# Autodesk Inventor assembly: a1614chal
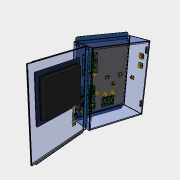
[picture p0: Inventor's stored thumbnail of the model, 180x180]
Saved by Autodesk Inventor 2020.1 (Build 241239000, 239)
## iProperties
Created: 2009-10-15
Part Number: a1614chal
Document SubType Name: Assembly
Designer: Thom Tremblay
Translation Standard: STEP AP214IS
FileName: a1614chal.STEP
PreProcessor: SolidWorks 2007
PostProcessor: Build: 253, Release: 2010 SP1 - Date: Wed 07/29/2009
Sent Units: inch
Uncertainty: 1e-05
Author: Thom Tremblay
## Documents named in this file (20)
- C:\Users\thom_tremblay\Desktop\Inventor ACP prep data\Week 1\Electrical Enclosure.iam
- C:\Users\thom_tremblay\Desktop\Inventor ACP prep data\Week 1\Electrical Enclosure\Clamp.ipt
- C:\Users\thom_tremblay\Desktop\Inventor ACP prep data\Week 1\Electrical Enclosure\Housing.iam
- C:\Users\thom_tremblay\Desktop\Inventor ACP prep data\Week 1\Electrical Enclosure\Panel_CHJunction_16x14.ipt
- C:\Users\thom_tremblay\Desktop\Inventor ACP prep data\Week 1\Electrical Enclosure\Cover.iam
- C:\Users\thom_tremblay\Desktop\Inventor ACP prep data\Week 1\Electrical Enclosure\Control Panel.ipt
- C:\Users\thom_tremblay\Desktop\Inventor ACP prep data\Week 1\Electrical Enclosure\Ribbon Tape.ipt
- C:\Users\thom_tremblay\Desktop\Inventor ACP prep data\Week 1\Electrical Enclosure\ribbon cable connector.ipt
- C:\Users\thom_tremblay\Desktop\Inventor ACP prep data\Week 1\Electrical Enclosure\Hinge.iam
- C:\Users\thom_tremblay\Desktop\Inventor ACP prep data\Week 1\Electrical Enclosure\Cable Mount.iam
- C:\Users\thom_tremblay\Desktop\Inventor ACP prep data\Week 1\Electrical Enclosure\Communication PCB.ipt
- C:\Users\thom_tremblay\Desktop\Inventor ACP prep data\Week 1\Electrical Enclosure\Graphics.iam
- C:\Users\thom_tremblay\Desktop\Inventor ACP prep data\Week 1\Electrical Enclosure\CPU_PCB.ipt
- C:\Users\thom_tremblay\Desktop\Inventor ACP prep data\Week 1\Electrical Enclosure\8 Pin Header.ipt
- C:\Users\thom_tremblay\Desktop\Inventor ACP prep data\Week 1\Electrical Enclosure\Connector, IDC, 8 Pin, SR.ipt
- C:\Users\thom_tremblay\Desktop\Inventor ACP prep data\Week 1\Electrical Enclosure\360124.ipt
- C:\Users\thom_tremblay\Desktop\Inventor ACP prep data\Week 1\Electrical Enclosure\12 Pin DR.ipt
- C:\Users\thom_tremblay\Desktop\Inventor ACP prep data\Week 1\Electrical Enclosure\RC Male Connector.ipt
- C:\Users\thom_tremblay\Desktop\Inventor ACP prep data\Week 1\Electrical Enclosure\DB9 Female.ipt
- C:\Users\thom_tremblay\Desktop\Inventor ACP prep data\Week 1\Electrical Enclosure\10 Pin DR.ipt
## Components (29 placed, 19 different names)
1. Clamp:1
2. Housing:1 [sub-assembly] — Insert:1, Angle:1, Mate:5, Mate:6, Mate:7, Flush:7, Mate:13, Mate:22, Flush:17, Flush:20, Insert:3, Angle:6, Mate:29, Flush:32
3. Panel_CHJunction_16x14:1 — Insert:1, Angle:1, Angle:2, Mate:15, Angle:4, Mate:17, Flush:8, Flush:9, Flush:10, Flush:11, Mate:18, Flush:12, Flush:13, Mate:30, Flush:33, Mate:32, Mate:34
4. Clamp:2
5. Hinge:1 [sub-assembly] — Mate:16
6. Cover:1 [sub-assembly] — Flush:3, Mate:2, Mate:3, Mate:4, Mate:14, Angle:3
7. Control Panel:1 — Flush:3, Mate:2, Mate:3, Mate:9, Mate:10, Mate:11, Mate:28, Flush:30, Flush:31
8. Ribbon Tape:1 — Mate:5, Mate:6, Flush:4, Mate:7
9. Ribbon Tape:2 — Mate:4, Flush:4, Flush:7
10. ribbon cable connector:1 — Mate:9, Mate:10, Mate:11
11. Communication PCB:1 — Mate:15, Angle:4, Flush:10, Flush:11, Flush:21, Flush:22, Mate:25, Flush:25, Flush:26
12. DB9 Female:1
13. RC Male Connector:1
14. Graphics:1 [sub-assembly] — Mate:17, Flush:8, Flush:9, Mate:31, Flush:34, Flush:35
15. CPU_PCB:1 — Mate:18, Flush:12, Flush:13, Mate:19, Flush:14, Flush:15, Mate:33
16. 8 Pin Header:1 — Mate:19, Flush:14, Flush:15, Flush:16, Mate:21
17. Connector, IDC, 8 Pin, SR:1 — Flush:16, Mate:21
18. 360124:1 — Mate:22, Flush:17, Flush:20
19. 360124:2 — Insert:3, Angle:6
20. 12 Pin DR:2 — Mate:25, Flush:25, Flush:26
21. 10 Pin DR:2 — Flush:21, Flush:22
22. 10 Pin DR:1 — Mate:31, Flush:34, Flush:35
23. DB9 Female:2 — Mate:28, Flush:30, Flush:31
24. Cable Mount:1 [sub-assembly] — Mate:13, Angle:2
25. Cable Mount:2 [sub-assembly] — Mate:14, Angle:3, Mate:16
26. Cable Mount:3 [sub-assembly] — Mate:29, Flush:32
27. Cable Mount:4 [sub-assembly] — Mate:30, Flush:33
28. Cable Mount:5 [sub-assembly] — Mate:32, Mate:33, Flush:36
29. Cable Mount:6 [sub-assembly] — Mate:34, Flush:36
## Relationships (73: Mate 33, Flush 32, Angle 6, Insert 2)
- [Mate]: Housing:1 ↔ Hinge:1
- [Flush] (-13.97 mm): Housing:1 ↔ Hinge:1
- [Flush] (121.2342 mm): Housing:1 ↔ Hinge:1
- Flush:3: Cover:1 ↔ Control Panel:1
- Mate:2: Cover:1 ↔ Control Panel:1
- Mate:3: Cover:1 ↔ Control Panel:1
- Insert:1: Housing:1 ↔ Panel_CHJunction_16x14:1
- Angle:1 (0 deg): Housing:1 ↔ Panel_CHJunction_16x14:1
- Mate:4: Cover:1 ↔ Ribbon Tape:2
- Mate:5: Housing:1 ↔ Ribbon Tape:1
- Mate:6 (50.8 mm): Housing:1 ↔ Ribbon Tape:1
- Flush:4: Ribbon Tape:1 ↔ Ribbon Tape:2
- Mate:7 (50.8 mm): Housing:1 ↔ Ribbon Tape:1
- [Mate] (63.5 mm): Hinge:1 ↔ Ribbon Tape:2
- Mate:9: Control Panel:1 ↔ ribbon cable connector:1
- Mate:10 (0.127 mm): Control Panel:1 ↔ ribbon cable connector:1
- Mate:11: Control Panel:1 ↔ ribbon cable connector:1
- [Mate]: Hinge:1 ↔ Cover:1
- [Flush] (12.446 mm): Hinge:1 ↔ Cover:1
- [Flush] (-0.7874 mm): Hinge:1 ↔ Cover:1
- Flush:7: Housing:1 ↔ Ribbon Tape:2
- Mate:13: Housing:1 ↔ Cable Mount:1
- Angle:2 (0 deg): Panel_CHJunction_16x14:1 ↔ Cable Mount:1
- Mate:14: Cover:1 ↔ Cable Mount:2
- Angle:3 (0 deg): Cover:1 ↔ Cable Mount:2
- Mate:15 (2.54 mm): Panel_CHJunction_16x14:1 ↔ Communication PCB:1
- Angle:4 (-90 deg): Panel_CHJunction_16x14:1 ↔ Communication PCB:1
- Mate:16 (50.8 mm): Hinge:1 ↔ Cable Mount:2
- Mate:17 (2.54 mm): Panel_CHJunction_16x14:1 ↔ Graphics:1
- Flush:8 (-15.24 mm): Panel_CHJunction_16x14:1 ↔ Graphics:1
- Flush:9 (-25.4 mm): Panel_CHJunction_16x14:1 ↔ Graphics:1
- Flush:10 (12.7 mm): Panel_CHJunction_16x14:1 ↔ Communication PCB:1
- Flush:11 (76.2 mm): Panel_CHJunction_16x14:1 ↔ Communication PCB:1
- Mate:18 (2.54 mm): Panel_CHJunction_16x14:1 ↔ CPU_PCB:1
- Flush:12 (50.8 mm): Panel_CHJunction_16x14:1 ↔ CPU_PCB:1
- Flush:13 (203.2 mm): Panel_CHJunction_16x14:1 ↔ CPU_PCB:1
- Mate:19: CPU_PCB:1 ↔ 8 Pin Header:1
- Flush:14 (1.27 mm): CPU_PCB:1 ↔ 8 Pin Header:1
- Flush:15 (21.59 mm): CPU_PCB:1 ↔ 8 Pin Header:1
- [Mate]: 8 Pin Header:1 ↔ Connector, IDC, 8 Pin, SR:1
- Flush:16: 8 Pin Header:1 ↔ Connector, IDC, 8 Pin, SR:1
- Mate:21: 8 Pin Header:1 ↔ Connector, IDC, 8 Pin, SR:1
- Mate:22: Housing:1 ↔ 360124:1
- Flush:17 (38.1 mm): Housing:1 ↔ 360124:1
- Flush:20 (76.2 mm): Housing:1 ↔ 360124:1
- Insert:3: Housing:1 ↔ 360124:2
- Angle:6 (0 deg): Housing:1 ↔ 360124:2
- Flush:21: Communication PCB:1 ↔ 10 Pin DR:2
- [Mate]: Communication PCB:1 ↔ 10 Pin DR:2
- Flush:22: Communication PCB:1 ↔ 10 Pin DR:2
- Mate:25: Communication PCB:1 ↔ 12 Pin DR:2
- Flush:25: Communication PCB:1 ↔ 12 Pin DR:2
- Flush:26: Communication PCB:1 ↔ 12 Pin DR:2
- [Mate]: RC Male Connector:1 ↔ Graphics:1
- [Angle] (0 deg): RC Male Connector:1 ↔ Graphics:1
- [Flush] (6.35 mm): RC Male Connector:1 ↔ Graphics:1
- [Flush] (-38.1 mm): RC Male Connector:1 ↔ Graphics:1
- [Flush] (-5.08 mm): DB9 Female:1 ↔ Graphics:1
- [Mate] (7.62 mm): DB9 Female:1 ↔ Graphics:1
- Mate:28: Control Panel:1 ↔ DB9 Female:2
- Flush:30 (5.08 mm): Control Panel:1 ↔ DB9 Female:2
- Flush:31 (16.51 mm): Control Panel:1 ↔ DB9 Female:2
- Mate:29: Housing:1 ↔ Cable Mount:3
- Flush:32 (88.9 mm): Housing:1 ↔ Cable Mount:3
- Mate:30: Panel_CHJunction_16x14:1 ↔ Cable Mount:4
- Flush:33 (127 mm): Panel_CHJunction_16x14:1 ↔ Cable Mount:4
- Mate:31: Graphics:1 ↔ 10 Pin DR:1
- Flush:34: Graphics:1 ↔ 10 Pin DR:1
- Flush:35: Graphics:1 ↔ 10 Pin DR:1
- Mate:32: Panel_CHJunction_16x14:1 ↔ Cable Mount:5
- Mate:33 (25.4 mm): CPU_PCB:1 ↔ Cable Mount:5
- Mate:34: Panel_CHJunction_16x14:1 ↔ Cable Mount:6
- Flush:36: Cable Mount:5 ↔ Cable Mount:6
## Named parameters: d17_d0 = 0 mm, d18_d1 = 12.446 mm, d19_d2 = -0.7874 mm, d64_d10 = 6.35 mm, d65_d11 = -38.1 mm, d66_d12 = -5.08 mm, d67_d13 = 7.62 mm, d68_d1 = 0 mm, d69_d3 = 0 deg
